# Autodesk Inventor assembly: Tensionador-4-Cabos_Modelo1
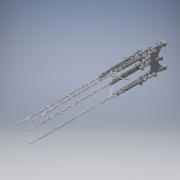
[picture p0: Inventor's stored thumbnail of the model, 180x180]
Saved by Autodesk Inventor 2018 (Build 220112000, 112)
## iProperties
Created: 2021-08-02
Part Number: Tensionador-4-Cabos_Modelo1
Document SubType Name: Assembly
Designer: L08619
Author: L08619
## Documents named in this file (5)
- C:\Users\l08619\Documents\Projetos\TAESA\Modelo 3D - Tensionadores e Suspensão\Tensionador\Tensionador-4-Cabos_Modelo1.iam
- C:\Users\l08619\Documents\Projetos\TAESA\Modelo 3D - Tensionadores e Suspensão\Tensionador\Balancim_4-Cabos_Modelo1.ipt
- C:\Users\l08619\Documents\Projetos\TAESA\Modelo 3D - Tensionadores e Suspensão\Tensionador\Clevis-Socket.iam
- C:\Users\l08619\Documents\Projetos\TAESA\Modelo 3D - Tensionadores e Suspensão\Tensionador\gpghmb32.iam
- C:\Users\l08619\Documents\Projetos\TAESA\Modelo 3D - Tensionadores e Suspensão\Tensionador\OPGW Tension set.iam
## Components (16 placed, 4 different names)
1. Balancim_4-Cabos_Modelo1:1 — Mate:1, Mate:2, Cylindrical:1, Cylindrical:2, Cylindrical:3, Cylindrical:4, Cylindrical:5, Cylindrical:6, Mate:3, Mate:4, Mate:5, Mate:6, Mate:7, Mate:8, Mate:9, Cylindrical:7
2. Clevis-Socket:1 [sub-assembly] — Cylindrical:1, Mate:3
3. Clevis-Socket:2 [sub-assembly] — Cylindrical:3, Mate:5
4. Clevis-Socket:3 [sub-assembly] — Cylindrical:2, Mate:4
5. gpghmb32:1 [sub-assembly] — Cylindrical:6, Mate:8
6. gpghmb32:2 [sub-assembly] — Cylindrical:5, Mate:6
7. gpghmb32:3 [sub-assembly] — Cylindrical:4, Mate:7
8. gpghmb32:4 [sub-assembly] — Mate:9, Cylindrical:7
9. gpghmb32:5 [sub-assembly] — Rotational:1, Angle:1, Mate:11
10. gpghmb32:6 [sub-assembly] — Angle:2, Mate:10, Rotational:2
11. gpghmb32:7 [sub-assembly] — Rotational:3
12. gpghmb32:8 [sub-assembly] — Cylindrical:8
13. OPGW Tension set:1 [sub-assembly] — Rotational:1
14. OPGW Tension set:2 [sub-assembly] — Rotational:2
15. OPGW Tension set:3 [sub-assembly] — Rotational:3
16. OPGW Tension set:4 [sub-assembly] — Cylindrical:8
## Relationships (24: Mate 11, CylindricalJoint 8, RevoluteJoint 3, Angle 2)
- Mate:1: Balancim_4-Cabos_Modelo1:1
- Mate:2: Balancim_4-Cabos_Modelo1:1
- Cylindrical:1: Balancim_4-Cabos_Modelo1:1 ↔ Clevis-Socket:1
- Cylindrical:2: Balancim_4-Cabos_Modelo1:1 ↔ Clevis-Socket:3
- Cylindrical:3: Balancim_4-Cabos_Modelo1:1 ↔ Clevis-Socket:2
- Cylindrical:4: Balancim_4-Cabos_Modelo1:1 ↔ gpghmb32:3
- Cylindrical:5: Balancim_4-Cabos_Modelo1:1 ↔ gpghmb32:2
- Cylindrical:6: Balancim_4-Cabos_Modelo1:1 ↔ gpghmb32:1
- Mate:3 (2 mm): Balancim_4-Cabos_Modelo1:1 ↔ Clevis-Socket:1
- Mate:4 (2 mm): Balancim_4-Cabos_Modelo1:1 ↔ Clevis-Socket:3
- Mate:5 (2 mm): Balancim_4-Cabos_Modelo1:1 ↔ Clevis-Socket:2
- Mate:6 (10 mm): Balancim_4-Cabos_Modelo1:1 ↔ gpghmb32:2
- Mate:7 (10 mm): Balancim_4-Cabos_Modelo1:1 ↔ gpghmb32:3
- Mate:8 (10 mm): Balancim_4-Cabos_Modelo1:1 ↔ gpghmb32:1
- Mate:9 (10 mm): Balancim_4-Cabos_Modelo1:1 ↔ gpghmb32:4
- Cylindrical:7: Balancim_4-Cabos_Modelo1:1 ↔ gpghmb32:4
- Rotational:1 [RevoluteJoint]: gpghmb32:5 ↔ OPGW Tension set:1
- Angle:1 (0 deg): gpghmb32:5
- Angle:2 (0 deg): gpghmb32:6
- Mate:10: gpghmb32:6
- Rotational:2 [RevoluteJoint]: gpghmb32:6 ↔ OPGW Tension set:2
- Mate:11: gpghmb32:5
- Rotational:3 [RevoluteJoint]: gpghmb32:7 ↔ OPGW Tension set:3
- Cylindrical:8: gpghmb32:8 ↔ OPGW Tension set:4
